# Autodesk Inventor assembly: Servo
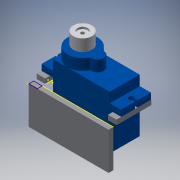
[picture p0: Inventor's stored thumbnail of the model, 180x180]
Saved by Autodesk Inventor 2016 (Build 200138000, 138)
## iProperties
Created: 2015-07-21
Part Number: Servo
Description: STEP AP214
Document SubType Name: Assembly
Designer: powasar16
Sending System: SolidWorks 2015
Preprocessor: SwSTEP 2.0
Title: TowPro-SG90-9g.STEP
Revision Number: ANY
## Documents named in this file (6)
- C:\Users\powasar16\Documents\GitHub\SpyderRobot\Inventor\Created Parts\Servo.iam
- C:\Users\powasar16\Documents\GitHub\SpyderRobot\Inventor\Imported Parts\STEP\Piece2.ipt
- C:\Users\powasar16\Documents\GitHub\SpyderRobot\Inventor\Imported Parts\STEP\Piece3.ipt
- C:\Users\powasar16\Documents\GitHub\SpyderRobot\Inventor\Imported Parts\STEP\Piece1.ipt
- C:\Users\powasar16\Documents\GitHub\SpyderRobot\Inventor\Imported Parts\STEP\A2.ipt
- C:\Users\powasar16\Documents\GitHub\SpyderRobot\Inventor\Created Parts\Servo_vice.ipt
## Components (5 placed, 5 different names)
1. Piece2_1 — Flush:2
2. Piece3_2
3. Piece1_3
4. A2_14
5. Servo_vice:1 — Flush:2
## Relationships (1: Flush 1)
- Flush:2 (3.175 mm): Piece2_1 ↔ Servo_vice:1
